# Autodesk Inventor assembly: COG_Evaluation
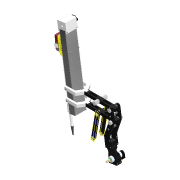
[picture p0: Inventor's stored thumbnail of the model, 180x180]
Saved by Autodesk Inventor 2022 (Build 260153000, 153)
## iProperties
Created: 2022-10-18
Part Number: COG_Evaluation
Document SubType Name: Assembly
Designer: alexw
Author: alexw
## Documents named in this file (18)
- C:\Users\alexw\Documents\Inventor\Projects\03_CurrentProjects\MasterThesis\PSM_V1_Rillenkugellager\COG\COG_Evaluation.iam
- C:\Users\alexw\Documents\Inventor\Projects\03_CurrentProjects\MasterThesis\PSM_V1_Rillenkugellager\ParallelMechanismus_Driven_Assembly_v2.1_Rillenkugellager_Anlaufscheibe.iam
- C:\Users\alexw\Documents\Inventor\Projects\03_CurrentProjects\MasterThesis\PSM_V1_Rillenkugellager\Adaptationhorizontalachse_obereGabel_Assembly_Rillenkugellager.iam
- C:\Users\alexw\Documents\Inventor\Projects\03_CurrentProjects\MasterThesis\PSM_V1_Rillenkugellager\Adaptationhorizontalachse_Assembly_Rillenkugellager.iam
- C:\Users\alexw\Documents\Inventor\Projects\03_CurrentProjects\MasterThesis\PSM_V1_Rillenkugellager\10_79_0000_0010_003.ipt
- C:\Users\alexw\Documents\Inventor\Projects\03_CurrentProjects\MasterThesis\PSM_V1_Rillenkugellager\circlips_din471_10_1.ipt
- C:\Users\alexw\Documents\Inventor\Projects\03_CurrentProjects\MasterThesis\PSM_V1_Rillenkugellager\din_988_10_x_16_x_0_10.ipt
- C:\Users\alexw\Documents\Inventor\Projects\03_CurrentProjects\MasterThesis\PSM_V1_Rillenkugellager\ParallelMechanismus_Support_Rillenkugellager.iam
- C:\Users\alexw\Documents\Inventor\Projects\03_CurrentProjects\MasterThesis\PSM_V1_Rillenkugellager\Maschinenbauteil\jtm-1018-010.ipt
- C:\Users\alexw\Documents\Inventor\Projects\03_CurrentProjects\MasterThesis\PSM_V1_Rillenkugellager\MorotFixation_CounterWeightHolder_Assembly.iam
- C:\Users\alexw\Documents\Inventor\Projects\03_CurrentProjects\MasterThesis\PSM_V1_Rillenkugellager\Ueberarbeiteter DaVincikopf\daVinci_Head_Assembly.iam
- C:\Users\alexw\Documents\Inventor\Projects\03_CurrentProjects\MasterThesis\PSM_V1_Rillenkugellager\Shaft_6mmx62mm.ipt
- C:\Users\alexw\Documents\Inventor\Projects\03_CurrentProjects\MasterThesis\PSM_V1_Rillenkugellager\SpringCompensation_Outside_SupportPart_Zwischenstueck.ipt
- C:\Users\alexw\Documents\Inventor\Projects\03_CurrentProjects\MasterThesis\PSM_V1_Rillenkugellager\ContentCenter\de-DE\ISO 4762(2)\ISO 4762 - M10 x 20ISO.ipt
- C:\Users\alexw\Documents\Inventor\Projects\03_CurrentProjects\MasterThesis\PSM_V1_Rillenkugellager\SpringCompensation_Innside_DrivenPart.ipt
- C:\Users\alexw\Documents\Inventor\Projects\03_CurrentProjects\MasterThesis\PSM_V1_Rillenkugellager\SpringCompensation_Innside_SupportPart.ipt
- C:\Users\alexw\Documents\Inventor\Projects\03_CurrentProjects\MasterThesis\PSM_V1_Rillenkugellager\SpringCompensation_Outside_DrivenPart.ipt
- C:\Users\alexw\Documents\Inventor\Projects\03_CurrentProjects\MasterThesis\PSM_V1_Rillenkugellager\SpringCompensation_Outside_SupportPart.ipt
## Components (34 placed, 17 different names)
1. ParallelMechanismus_Driven_Assembly_v2.1_Rillenkugellager_Anlaufscheibe:1 [sub-assembly] — Winkel:1, Passend:69, Passend:72
2. Adaptationhorizontalachse_obereGabel_Assembly_Rillenkugellager:1 [sub-assembly] — Winkel:1
3. Adaptationhorizontalachse_Assembly_Rillenkugellager:1 [sub-assembly]
4. 10_79_0000_0010_003:1
5. 10_79_0000_0010_003:2
6. 10_79_0000_0010_003:3
7. 10_79_0000_0010_003:4
8. circlips_din471_10_1:1
9. circlips_din471_10_1:2
10. din_988_10_x_16_x_0_10:1
11. din_988_10_x_16_x_0_10:2
12. din_988_10_x_16_x_0_10:3
13. din_988_10_x_16_x_0_10:4
14. circlips_din471_10_1:3
15. circlips_din471_10_1:4
16. ParallelMechanismus_Support_Rillenkugellager:1 [sub-assembly]
17. ParallelMechanismus_Support_Rillenkugellager:2 [sub-assembly] — Passend:68, Passend:71
18. jtm-1018-010:1
19. jtm-1018-010:2
20. MorotFixation_CounterWeightHolder_Assembly:1 [sub-assembly] — Passend:64, Passend:69, Passend:71
21. daVinci_Head_Assembly:1 [sub-assembly]
22. Shaft_6mmx62mm:1
23. SpringCompensation_Outside_SupportPart_Zwischenstueck:1
24. SpringCompensation_Outside_SupportPart_Zwischenstueck:2
25. ISO 4762 M10 x 20:1
26. ISO 4762 M10 x 20:2
27. SpringCompensation_Innside_DrivenPart:1
28. SpringCompensation_Innside_DrivenPart:2
29. SpringCompensation_Innside_SupportPart:1
30. SpringCompensation_Innside_SupportPart:2
31. SpringCompensation_Outside_DrivenPart:1
32. SpringCompensation_Outside_DrivenPart:2
33. SpringCompensation_Outside_SupportPart:1
34. SpringCompensation_Outside_SupportPart:2
## Relationships (78: Mate 72, Flush 5, Angle 1)
- [Mate]: 10_79_0000_0010_003:1 ↔ circlips_din471_10_1:1
- [Mate]: 10_79_0000_0010_003:2 ↔ circlips_din471_10_1:2
- [Mate]: 10_79_0000_0010_003:2 ↔ din_988_10_x_16_x_0_10:1
- [Mate]: Adaptationhorizontalachse_Assembly_Rillenkugellager:1 ↔ din_988_10_x_16_x_0_10:1
- [Mate]: circlips_din471_10_1:2 ↔ din_988_10_x_16_x_0_10:1
- [Mate]: 10_79_0000_0010_003:1 ↔ din_988_10_x_16_x_0_10:2
- [Mate]: Adaptationhorizontalachse_obereGabel_Assembly_Rillenkugellager:1 ↔ din_988_10_x_16_x_0_10:2
- [Mate]: circlips_din471_10_1:1 ↔ din_988_10_x_16_x_0_10:2
- [Mate]: 10_79_0000_0010_003:3 ↔ din_988_10_x_16_x_0_10:3
- [Mate]: Adaptationhorizontalachse_Assembly_Rillenkugellager:1 ↔ din_988_10_x_16_x_0_10:3
- [Mate]: 10_79_0000_0010_003:4 ↔ din_988_10_x_16_x_0_10:4
- [Mate]: Adaptationhorizontalachse_obereGabel_Assembly_Rillenkugellager:1 ↔ din_988_10_x_16_x_0_10:4
- [Mate]: 10_79_0000_0010_003:4 ↔ circlips_din471_10_1:3
- [Mate]: din_988_10_x_16_x_0_10:4 ↔ circlips_din471_10_1:3
- [Mate]: 10_79_0000_0010_003:3 ↔ circlips_din471_10_1:4
- [Mate]: din_988_10_x_16_x_0_10:3 ↔ circlips_din471_10_1:4
- [Mate]: ParallelMechanismus_Driven_Assembly_v2.1_Rillenkugellager_Anlaufscheibe:1 ↔ Adaptationhorizontalachse_obereGabel_Assembly_Rillenkugellager:1
- [Mate]: ParallelMechanismus_Driven_Assembly_v2.1_Rillenkugellager_Anlaufscheibe:1 ↔ Adaptationhorizontalachse_Assembly_Rillenkugellager:1
- [Mate]: ParallelMechanismus_Driven_Assembly_v2.1_Rillenkugellager_Anlaufscheibe:1 ↔ Adaptationhorizontalachse_obereGabel_Assembly_Rillenkugellager:1
- [Mate]: ParallelMechanismus_Driven_Assembly_v2.1_Rillenkugellager_Anlaufscheibe:1 ↔ Adaptationhorizontalachse_Assembly_Rillenkugellager:1
- [Mate]: ParallelMechanismus_Support_Rillenkugellager:2 ↔ jtm-1018-010:2
- [Mate]: ParallelMechanismus_Support_Rillenkugellager:1 ↔ jtm-1018-010:1
- [Mate]: ParallelMechanismus_Support_Rillenkugellager:1 ↔ ParallelMechanismus_Support_Rillenkugellager:2
- [Mate]: Adaptationhorizontalachse_obereGabel_Assembly_Rillenkugellager:1 ↔ 10_79_0000_0010_003:4
- [Mate]: Adaptationhorizontalachse_Assembly_Rillenkugellager:1 ↔ 10_79_0000_0010_003:3
- [Mate]: Adaptationhorizontalachse_obereGabel_Assembly_Rillenkugellager:1 ↔ 10_79_0000_0010_003:1
- [Mate]: Adaptationhorizontalachse_Assembly_Rillenkugellager:1 ↔ 10_79_0000_0010_003:2
- [Flush]: Adaptationhorizontalachse_obereGabel_Assembly_Rillenkugellager:1 ↔ 10_79_0000_0010_003:4
- [Flush]: Adaptationhorizontalachse_Assembly_Rillenkugellager:1 ↔ 10_79_0000_0010_003:3
- [Flush]: Adaptationhorizontalachse_obereGabel_Assembly_Rillenkugellager:1 ↔ 10_79_0000_0010_003:1
- [Flush]: Adaptationhorizontalachse_Assembly_Rillenkugellager:1 ↔ 10_79_0000_0010_003:2
- [Mate]: 10_79_0000_0010_003:1 ↔ daVinci_Head_Assembly:1
- [Mate]: 10_79_0000_0010_003:2 ↔ daVinci_Head_Assembly:1
- [Mate]: Adaptationhorizontalachse_obereGabel_Assembly_Rillenkugellager:1 ↔ daVinci_Head_Assembly:1
- [Mate]: ParallelMechanismus_Driven_Assembly_v2.1_Rillenkugellager_Anlaufscheibe:1 ↔ MorotFixation_CounterWeightHolder_Assembly:1
- [Mate]: ParallelMechanismus_Driven_Assembly_v2.1_Rillenkugellager_Anlaufscheibe:1 ↔ MorotFixation_CounterWeightHolder_Assembly:1
- [Mate]: ParallelMechanismus_Driven_Assembly_v2.1_Rillenkugellager_Anlaufscheibe:1 ↔ Shaft_6mmx62mm:1
- [Flush]: ParallelMechanismus_Driven_Assembly_v2.1_Rillenkugellager_Anlaufscheibe:1 ↔ Shaft_6mmx62mm:1
- [Mate]: Adaptationhorizontalachse_obereGabel_Assembly_Rillenkugellager:1 ↔ SpringCompensation_Outside_SupportPart_Zwischenstueck:1
- [Mate]: Adaptationhorizontalachse_obereGabel_Assembly_Rillenkugellager:1 ↔ SpringCompensation_Outside_SupportPart_Zwischenstueck:1
- [Mate]: Adaptationhorizontalachse_obereGabel_Assembly_Rillenkugellager:1 ↔ SpringCompensation_Outside_SupportPart_Zwischenstueck:2
- [Mate]: Adaptationhorizontalachse_obereGabel_Assembly_Rillenkugellager:1 ↔ SpringCompensation_Outside_SupportPart_Zwischenstueck:2
- [Mate]: Adaptationhorizontalachse_obereGabel_Assembly_Rillenkugellager:1 ↔ ISO 4762 M10 x 20:1
- [Mate]: SpringCompensation_Outside_SupportPart_Zwischenstueck:2 ↔ ISO 4762 M10 x 20:1
- [Mate]: Adaptationhorizontalachse_obereGabel_Assembly_Rillenkugellager:1 ↔ ISO 4762 M10 x 20:2
- [Mate]: SpringCompensation_Outside_SupportPart_Zwischenstueck:1 ↔ ISO 4762 M10 x 20:2
- [Mate]: ParallelMechanismus_Driven_Assembly_v2.1_Rillenkugellager_Anlaufscheibe:1 ↔ SpringCompensation_Innside_DrivenPart:1
- [Mate]: ParallelMechanismus_Driven_Assembly_v2.1_Rillenkugellager_Anlaufscheibe:1 ↔ SpringCompensation_Innside_DrivenPart:1
- [Mate]: ParallelMechanismus_Driven_Assembly_v2.1_Rillenkugellager_Anlaufscheibe:1 ↔ SpringCompensation_Innside_DrivenPart:2
- [Mate]: ParallelMechanismus_Driven_Assembly_v2.1_Rillenkugellager_Anlaufscheibe:1 ↔ SpringCompensation_Innside_DrivenPart:2
- [Mate]: ParallelMechanismus_Support_Rillenkugellager:1 ↔ SpringCompensation_Innside_SupportPart:1
- [Mate]: ParallelMechanismus_Support_Rillenkugellager:1 ↔ SpringCompensation_Innside_SupportPart:1
- [Mate]: ParallelMechanismus_Support_Rillenkugellager:2 ↔ SpringCompensation_Innside_SupportPart:2
- [Mate]: ParallelMechanismus_Support_Rillenkugellager:2 ↔ SpringCompensation_Innside_SupportPart:2
- [Mate]: ParallelMechanismus_Driven_Assembly_v2.1_Rillenkugellager_Anlaufscheibe:1 ↔ SpringCompensation_Outside_DrivenPart:1
- [Mate]: ParallelMechanismus_Driven_Assembly_v2.1_Rillenkugellager_Anlaufscheibe:1 ↔ SpringCompensation_Outside_DrivenPart:1
- [Mate]: ParallelMechanismus_Driven_Assembly_v2.1_Rillenkugellager_Anlaufscheibe:1 ↔ SpringCompensation_Outside_DrivenPart:2
- [Mate]: ParallelMechanismus_Driven_Assembly_v2.1_Rillenkugellager_Anlaufscheibe:1 ↔ SpringCompensation_Outside_DrivenPart:2
- [Mate]: SpringCompensation_Outside_SupportPart_Zwischenstueck:1 ↔ SpringCompensation_Outside_SupportPart:1
- [Mate]: SpringCompensation_Outside_SupportPart_Zwischenstueck:1 ↔ SpringCompensation_Outside_SupportPart:1
- [Mate]: SpringCompensation_Outside_SupportPart_Zwischenstueck:2 ↔ SpringCompensation_Outside_SupportPart:2
- [Mate]: SpringCompensation_Outside_SupportPart_Zwischenstueck:2 ↔ SpringCompensation_Outside_SupportPart:2
- [Mate]: Adaptationhorizontalachse_Assembly_Rillenkugellager:1 ↔ jtm-1018-010:1
- [Mate]: Adaptationhorizontalachse_Assembly_Rillenkugellager:1 ↔ jtm-1018-010:1
- [Mate]: Adaptationhorizontalachse_Assembly_Rillenkugellager:1 ↔ jtm-1018-010:2
- [Mate]: Adaptationhorizontalachse_Assembly_Rillenkugellager:1 ↔ jtm-1018-010:2
- [Mate]: Adaptationhorizontalachse_Assembly_Rillenkugellager:1 ↔ ParallelMechanismus_Support_Rillenkugellager:1
- [Mate]: Adaptationhorizontalachse_Assembly_Rillenkugellager:1 ↔ ParallelMechanismus_Support_Rillenkugellager:2
- Passend:64 [Mate]: MorotFixation_CounterWeightHolder_Assembly:1
- Winkel:1 [Angle] (-8.48 deg): ParallelMechanismus_Driven_Assembly_v2.1_Rillenkugellager_Anlaufscheibe:1 ↔ Adaptationhorizontalachse_obereGabel_Assembly_Rillenkugellager:1
- Passend:65 [Mate]
- Passend:66 [Mate]
- Passend:67 [Mate]
- Passend:68 [Mate]: ParallelMechanismus_Support_Rillenkugellager:2
- Passend:69 [Mate]: ParallelMechanismus_Driven_Assembly_v2.1_Rillenkugellager_Anlaufscheibe:1 ↔ MorotFixation_CounterWeightHolder_Assembly:1
- Passend:70 [Mate]
- Passend:71 [Mate] (100 mm): ParallelMechanismus_Support_Rillenkugellager:2 ↔ MorotFixation_CounterWeightHolder_Assembly:1
- Passend:72 [Mate]: ParallelMechanismus_Driven_Assembly_v2.1_Rillenkugellager_Anlaufscheibe:1
